# Autodesk Inventor assembly: FullFrame
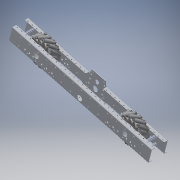
[picture p0: Inventor's stored thumbnail of the model, 180x180]
Saved by Autodesk Inventor 2019 (Build 230136000, 136)
## iProperties
Created: 2019-01-09
Part Number: FullFrame
Document SubType Name: Assembly
Designer: james
Author: james
## Documents named in this file (5)
- F:\JimsDesign\2019CHS4089\FullFrame.iam
- F:\JimsDesign\Library\AndyMark\am-3922 AM14U4 Inside Plate.ipt
- F:\JimsDesign\Library\AndyMark\am-3921 AM14U4 Outside Plate.ipt
- F:\JimsDesign\Library\AndyMark\3.375in Churro.ipt
- F:\JimsDesign\Library\AndyMark\am-3479L 6 SR Mecanum Left.iam
## Components (8 placed, 4 different names)
1. am-3922 AM14U4 Inside Plate:1 — Mate:9, Mate:10, Mate:11
2. am-3921 AM14U4 Outside Plate:1 — Mate:1, Mate:2, Mate:3, Mate:4, Mate:5, Mate:6, Mate:7, Mate:8, Mate:12, Mate:13
3. 3.375in Churro:1 — Mate:7, Mate:8, Mate:11
4. 3.375in Churro:2 — Mate:1, Mate:2, Mate:9, Mate:10
5. 3.375in Churro:3 — Mate:3, Mate:4
6. 3.375in Churro:4 — Mate:5, Mate:6
7. am-3479L 6 SR Mecanum Left:1 [sub-assembly] — Mate:12, Flush:1
8. am-3479L 6 SR Mecanum Left:2 [sub-assembly] — Flush:1, Mate:13
## Relationships (14: Mate 13, Flush 1)
- Mate:1: am-3921 AM14U4 Outside Plate:1 ↔ 3.375in Churro:2
- Mate:2: am-3921 AM14U4 Outside Plate:1 ↔ 3.375in Churro:2
- Mate:3: am-3921 AM14U4 Outside Plate:1 ↔ 3.375in Churro:3
- Mate:4: am-3921 AM14U4 Outside Plate:1 ↔ 3.375in Churro:3
- Mate:5: am-3921 AM14U4 Outside Plate:1 ↔ 3.375in Churro:4
- Mate:6: am-3921 AM14U4 Outside Plate:1 ↔ 3.375in Churro:4
- Mate:7: am-3921 AM14U4 Outside Plate:1 ↔ 3.375in Churro:1
- Mate:8: am-3921 AM14U4 Outside Plate:1 ↔ 3.375in Churro:1
- Mate:9: am-3922 AM14U4 Inside Plate:1 ↔ 3.375in Churro:2
- Mate:10: am-3922 AM14U4 Inside Plate:1 ↔ 3.375in Churro:2
- Mate:11: am-3922 AM14U4 Inside Plate:1 ↔ 3.375in Churro:1
- Mate:12: am-3921 AM14U4 Outside Plate:1 ↔ am-3479L 6 SR Mecanum Left:1
- Flush:1: am-3479L 6 SR Mecanum Left:1 ↔ am-3479L 6 SR Mecanum Left:2
- Mate:13: am-3921 AM14U4 Outside Plate:1 ↔ am-3479L 6 SR Mecanum Left:2
